# Autodesk Inventor assembly: Raumluftsensor
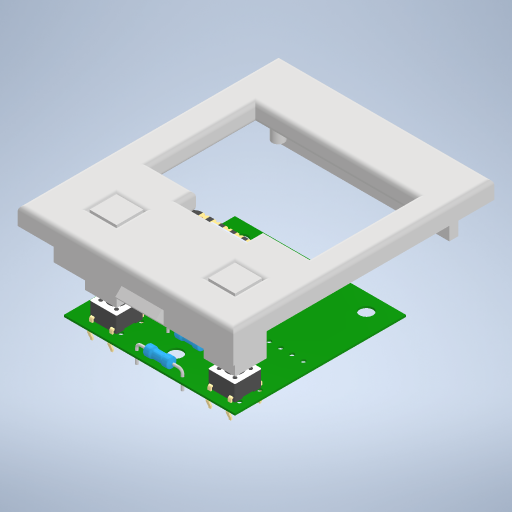
[picture p0: Inventor's stored thumbnail of the model, 512x512]
Saved by Autodesk Inventor 2024 (Build 280153000, 153)
## iProperties
Created: 2025-04-30
Part Number: Raumluftsensor
Document SubType Name: Assembly
Designer: tobia
Author: tobia
## Documents named in this file (7)
- S:\HTL-Anichstrasse\4.Klasse\PBE\KuenC\RaumluftsensorC3\Raumluftsensor.iam
- S:\HTL-Anichstrasse\4.Klasse\PBE\KuenC\RaumluftsensorC3\RaumluftsensorC3.ipt
- S:\HTL-Anichstrasse\4.Klasse\PBE\KuenC\RaumluftsensorC3\Unterseite.ipt
- S:\HTL-Anichstrasse\4.Klasse\PBE\KuenC\1-3-oled-display-128x64-1.snapshot.5\stp\AZ-Delivery - OLED13 IIC\AZ-Delivery - OLED13 IIC.ipt
- S:\HTL-Anichstrasse\4.Klasse\PBE\KuenC\gy-bme280-1.snapshot.4\GY-BME280\GY-BME280.ipt
- S:\HTL-Anichstrasse\4.Klasse\PBE\KuenC\RaumluftsensorC3\Deckel.ipt
- S:\HTL-Anichstrasse\4.Klasse\PBE\KuenC\RaumluftsensorC3\Taster.ipt
## Components (6 placed, 6 different names)
1. Unterseite:1 — Drehbar:1, Fluchtend:1
2. RaumluftsensorC3:1 — Drehbar:1
3. AZ-Delivery - OLED13 IIC:1
4. GY-BME280:1
5. Deckel:1 — Fluchtend:1, Fluchtend:2
6. Taster:1 — Fluchtend:2
## Relationships (3: Flush 2, RevoluteJoint 1)
- Drehbar:1 [RevoluteJoint]: Unterseite:1 ↔ RaumluftsensorC3:1
- Fluchtend:1 [Flush]: Unterseite:1 ↔ Deckel:1
- Fluchtend:2 [Flush]: Deckel:1 ↔ Taster:1
